# Autodesk Inventor assembly: Lamp
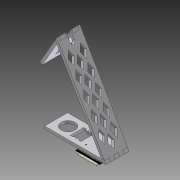
[picture p0: Inventor's stored thumbnail of the model, 180x180]
Saved by Autodesk Inventor 2012 SP2 (Build 160219200, 219)
## iProperties
Created: 2013-02-09
Part Number: Lamp
Document SubType Name: Assembly
Designer: blacki
Author: blacki
## Documents named in this file (7)
- E:\PROJEKTE\WELTHERRSCHAFT\04_SENSELAMP\FRAME\ANGLEDFRAME\Lamp.iam
- E:\PROJEKTE\WELTHERRSCHAFT\04_SENSELAMP\FRAME\ANGLEDFRAME\TriangleBase.ipt
- E:\PROJEKTE\WELTHERRSCHAFT\04_SENSELAMP\FRAME\ANGLEDFRAME\TriangleLongLeg.ipt
- E:\PROJEKTE\WELTHERRSCHAFT\04_SENSELAMP\FRAME\ANGLEDFRAME\TriangleShortLeg.ipt
- E:\PROJEKTE\WELTHERRSCHAFT\04_SENSELAMP\FRAME\ANGLEDFRAME\board_image.ipt
- E:\PROJEKTE\WELTHERRSCHAFT\04_SENSELAMP\FRAME\ANGLEDFRAME\TLwr703n_image.ipt
- E:\PROJEKTE\WELTHERRSCHAFT\04_SENSELAMP\FRAME\ANGLEDFRAME\PcbSpacer.ipt
## Components (7 placed, 6 different names)
1. TriangleBase:1 — Flush:2, Angle:1, Mate:1, Mate:3, Mate:6, Flush:5, Mate:17, Flush:9
2. TriangleLongLeg:1 — Flush:1, Flush:2, Angle:1, Angle:2, Mate:1, Flush:3, Flush:4
3. TriangleShortLeg:1 — Flush:1, Angle:2, Flush:3, Flush:4
4. board_image:1 — Mate:4, Mate:5, Mate:6, Flush:5, Flush:6, Flush:7, Mate:7, Mate:8, Mate:9, Flush:9
5. TLwr703n_image:1 — Mate:3, Mate:4, Mate:5, Flush:6, Mate:17
6. PcbSpacer:1 — Flush:7, Mate:7
7. PcbSpacer:2 — Mate:8, Mate:9
## Relationships (19: Mate 9, Flush 8, Angle 2)
- Flush:1: TriangleLongLeg:1 ↔ TriangleShortLeg:1
- Flush:2: TriangleBase:1 ↔ TriangleLongLeg:1
- Angle:1 (120 deg): TriangleBase:1 ↔ TriangleLongLeg:1
- Angle:2 (60 deg): TriangleLongLeg:1 ↔ TriangleShortLeg:1
- Mate:1: TriangleBase:1 ↔ TriangleLongLeg:1
- Flush:3: TriangleLongLeg:1 ↔ TriangleShortLeg:1
- Flush:4: TriangleLongLeg:1 ↔ TriangleShortLeg:1
- Mate:3: TriangleBase:1 ↔ TLwr703n_image:1
- Mate:4 (10 mm): board_image:1 ↔ TLwr703n_image:1
- Mate:5: board_image:1 ↔ TLwr703n_image:1
- Mate:6 (10 mm): TriangleBase:1 ↔ board_image:1
- Flush:5: TriangleBase:1 ↔ board_image:1
- Flush:6: board_image:1 ↔ TLwr703n_image:1
- Flush:7: board_image:1 ↔ PcbSpacer:1
- Mate:7: board_image:1 ↔ PcbSpacer:1
- Mate:8: board_image:1 ↔ PcbSpacer:2
- Mate:9: board_image:1 ↔ PcbSpacer:2
- Mate:17 (10 mm): TriangleBase:1 ↔ TLwr703n_image:1
- Flush:9: TriangleBase:1 ↔ board_image:1
